# Autodesk Inventor assembly: arm_assy_v1
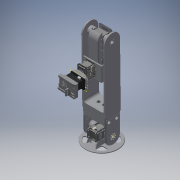
[picture p0: Inventor's stored thumbnail of the model, 180x180]
Saved by Autodesk Inventor 2018 (Build 220112000, 112)
## iProperties
Created: 2018-03-06
Part Number: arm_assy_v1
Document SubType Name: Assembly
Designer: Matthew
Author: Matthew
## Documents named in this file (11)
- C:\Users\mshaw2\OneDrive - University of Plymouth\ROCO224\arm_assy_v1.iam
- C:\Users\mshaw2\OneDrive - University of Plymouth\ROCO224\base_turret_v1.ipt
- C:\Users\mshaw2\OneDrive - University of Plymouth\ROCO224\ENS_SERVO-RX-28.iam
- C:\Users\mshaw2\OneDrive - University of Plymouth\ROCO224\arm_segment_1_1a.ipt
- C:\Users\mshaw2\OneDrive - University of Plymouth\ROCO224\arm_segment_1_1b.ipt
- C:\Users\mshaw2\OneDrive - University of Plymouth\ROCO224\arm_segment_1_2a.ipt
- C:\Users\mshaw2\OneDrive - University of Plymouth\ROCO224\arm_segment_1_2b.ipt
- C:\Users\mshaw2\OneDrive - University of Plymouth\ROCO224\arm_segment_2_1.ipt
- C:\Users\mshaw2\OneDrive - University of Plymouth\ROCO224\arm_segment_3_1.ipt
- C:\Users\mshaw2\OneDrive - University of Plymouth\ROCO224\grabber_rotating_mount_1.ipt
- C:\Users\mshaw2\OneDrive - University of Plymouth\ROCO224\Grabber_Assy.iam
## Components (14 placed, 10 different names)
1. base_turret_v1:1 — Rigid:1
2. ENS_SERVO-RX-28:1 [sub-assembly] — Rigid:1, Rotational:1
3. arm_segment_1_1a:1 — Rotational:1, Rigid:2, Rigid:3
4. arm_segment_1_1b:1 — Rigid:2
5. arm_segment_1_2a:1 — Rigid:3, Rigid:4, Rotational:2
6. arm_segment_1_2b:1 — Rigid:4, Angle:1
7. ENS_SERVO-RX-28:2 [sub-assembly] — Rotational:2, Rigid:6
8. arm_segment_2_1:1 — Rigid:5, Angle:1
9. arm_segment_2_1:2 — Rigid:5, Rigid:6, Rigid:7, Angle:2
10. ENS_SERVO-RX-28:3 [sub-assembly] — Rigid:7, Rotational:3
11. arm_segment_3_1:1 — Rotational:3, Angle:2, Rigid:8
12. ENS_SERVO-RX-28:4 [sub-assembly] — Rigid:8, Rotational:4
13. grabber_rotating_mount_1:1 — Rotational:4, Rigid:9
14. Grabber_Assy:1 [sub-assembly] — Rigid:9
## Relationships (15: WeldJoint 9, RevoluteJoint 4, Angle 2)
- Rigid:1 [WeldJoint]: base_turret_v1:1 ↔ ENS_SERVO-RX-28:1
- Rotational:1 [RevoluteJoint] (0.5 mm): ENS_SERVO-RX-28:1 ↔ arm_segment_1_1a:1
- Rigid:2 [WeldJoint]: arm_segment_1_1a:1 ↔ arm_segment_1_1b:1
- Rigid:3 [WeldJoint] (0.3 mm): arm_segment_1_1a:1 ↔ arm_segment_1_2a:1
- Rigid:4 [WeldJoint]: arm_segment_1_2a:1 ↔ arm_segment_1_2b:1
- Rotational:2 [RevoluteJoint] (-0.5 mm): arm_segment_1_2a:1 ↔ ENS_SERVO-RX-28:2
- Rigid:5 [WeldJoint] (0.5 mm): arm_segment_2_1:1 ↔ arm_segment_2_1:2
- Rigid:6 [WeldJoint]: ENS_SERVO-RX-28:2 ↔ arm_segment_2_1:2
- Rigid:7 [WeldJoint]: arm_segment_2_1:2 ↔ ENS_SERVO-RX-28:3
- Rotational:3 [RevoluteJoint] (1 mm): ENS_SERVO-RX-28:3 ↔ arm_segment_3_1:1
- Angle:1 (0 deg): arm_segment_1_2b:1 ↔ arm_segment_2_1:1
- Angle:2 (90 deg): arm_segment_2_1:2 ↔ arm_segment_3_1:1
- Rigid:8 [WeldJoint]: arm_segment_3_1:1 ↔ ENS_SERVO-RX-28:4
- Rotational:4 [RevoluteJoint]: ENS_SERVO-RX-28:4 ↔ grabber_rotating_mount_1:1
- Rigid:9 [WeldJoint]: grabber_rotating_mount_1:1 ↔ Grabber_Assy:1
